# Autodesk Inventor assembly: Assembly_miniSPIM_v1
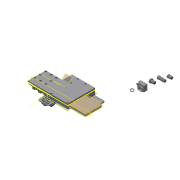
[picture p0: Inventor's stored thumbnail of the model, 180x180]
Saved by Autodesk Inventor 2019 (Build 230136000, 136)
## iProperties
Created: 2019-10-10
Part Number: Assembly_miniSPIM_v1
Document SubType Name: Assembly
Designer: diederichbenedict
Author: diederichbenedict
## Documents named in this file (19)
- C:\Users\diederichbenedict\Dropbox\Dokumente\Promotion\PROJECTS\miniSPIM\INVENTOR\Assembly_miniSPIM_v1.iam
- C:\Users\diederichbenedict\Dropbox\Dokumente\Promotion\PROJECTS\miniSPIM\INVENTOR\00_Huawei_P9.ipt
- C:\Users\diederichbenedict\Dropbox\Dokumente\Promotion\PROJECTS\miniSPIM\INVENTOR\00_Lens_f_25mm.ipt
- C:\Users\diederichbenedict\Dropbox\Dokumente\Promotion\PROJECTS\miniSPIM\INVENTOR\00_Sony_MDL_Projector.ipt
- C:\Users\diederichbenedict\Dropbox\Dokumente\Promotion\PROJECTS\miniSPIM\INVENTOR\00_XY_stage-CHUO_SEIKI_LD-647-R1.iam
- C:\Users\diederichbenedict\Dropbox\Dokumente\Promotion\PROJECTS\miniSPIM\INVENTOR\101_CCTV_Lens_Thread.ipt
- C:\Users\diederichbenedict\Dropbox\Dokumente\Promotion\PROJECTS\miniSPIM\INVENTOR\102_Z_Focus_CCTV_Camera.ipt
- C:\Users\diederichbenedict\Dropbox\Dokumente\Promotion\PROJECTS\miniSPIM\INVENTOR\103_CCTV_Lens_f2.8_f#1.ipt
- C:\Users\diederichbenedict\Dropbox\Dokumente\Promotion\PROJECTS\miniSPIM\INVENTOR\104_CCTV_Lens_f2.8_#1.ipt
- C:\Users\diederichbenedict\Dropbox\Dokumente\Promotion\PROJECTS\miniSPIM\INVENTOR\105_CCTV_Lens_f6_f#1.ipt
- C:\Users\diederichbenedict\Dropbox\Dokumente\Promotion\PROJECTS\miniSPIM\INVENTOR\00_Lightpath.ipt
- C:\Users\diederichbenedict\Dropbox\Dokumente\Promotion\PROJECTS\miniSPIM\INVENTOR\10_MiniSPIM_Base_v1.ipt
- C:\Users\diederichbenedict\Dropbox\Dokumente\Promotion\PROJECTS\miniSPIM\INVENTOR\00_Mirror_10mmDia.ipt
- C:\Users\diederichbenedict\Dropbox\Dokumente\Promotion\PROJECTS\miniSPIM\INVENTOR\10_MiniSPIM_Lid.ipt
- C:\Users\diederichbenedict\Dropbox\Dokumente\Promotion\PROJECTS\miniSPIM\INVENTOR\10_MiniSPIM_Smarthponebase.ipt
- C:\Users\diederichbenedict\Dropbox\Dokumente\Promotion\PROJECTS\miniSPIM\INVENTOR\10_MiniSPIM_Samplechamber.ipt
- C:\Users\diederichbenedict\Dropbox\Dokumente\Promotion\PROJECTS\miniSPIM\INVENTOR\10_MiniSPIM_Sampleholder.ipt
- C:\Users\diederichbenedict\Dropbox\Dokumente\Promotion\PROJECTS\miniSPIM\INVENTOR\00_XY-Tisch_Chinaware_Benedict-Diederich.ipt
- C:\Users\diederichbenedict\Dropbox\Dokumente\Promotion\PROJECTS\miniSPIM\INVENTOR\10_MiniSPIM_XY_Stageplate.ipt
## Components (19 placed, 18 different names)
1. 00_Huawei_P9:1 — Mate:1, Angle:1, Mate:2
2. 00_Lens_f_25mm:1 — Insert:1, Flush:4
3. 00_Sony_MDL_Projector:1 — Flush:1, Mate:1, Angle:1, Angle:2, Insert:1, Flush:3, Flush:5, Flush:6, Flush:9, Flush:10
4. 00_XY_stage-CHUO_SEIKI_LD-647-R1:1 [sub-assembly] — Flush:1, Angle:2, Flush:8, Flush:17, Flush:18, Mate:6, Mate:7, Flush:20, Flush:21
5. 101_CCTV_Lens_Thread:1
6. 102_Z_Focus_CCTV_Camera:1
7. 103_CCTV_Lens_f2.8_f#1:1
8. 104_CCTV_Lens_f2.8_#1:1
9. 105_CCTV_Lens_f6_f#1:1
10. 103_CCTV_Lens_f2.8_f#1:2 — Mate:3, Flush:7
11. 00_Lightpath:1 — Flush:3, Flush:4, Flush:5, Flush:6, Mate:2, Mate:3, Flush:7, Flush:8, Mate:4, Angle:3
12. 10_MiniSPIM_Base_v1:1 — Flush:9, Flush:10, Flush:11, Flush:12, Flush:15, Flush:16, Flush:19
13. 00_Mirror_10mmDia:1 — Mate:5
14. 10_MiniSPIM_Lid:1 — Flush:11, Flush:12, Flush:13, Flush:14
15. 10_MiniSPIM_Smarthponebase:1 — Flush:13, Flush:14
16. 10_MiniSPIM_Samplechamber:1 — Flush:15, Flush:16
17. 10_MiniSPIM_Sampleholder:1 — Flush:17, Flush:18
18. 00_XY-Tisch_Chinaware_Benedict-Diederich:1 — Mate:6, Flush:19, Mate:7
19. 10_MiniSPIM_XY_Stageplate:1 — Flush:20, Flush:21
## Relationships (31: Flush 20, Mate 7, Angle 3, Insert 1)
- Flush:1: 00_Sony_MDL_Projector:1 ↔ 00_XY_stage-CHUO_SEIKI_LD-647-R1:1
- Mate:1 (10 mm): 00_Huawei_P9:1 ↔ 00_Sony_MDL_Projector:1
- Angle:1 (0 deg): 00_Huawei_P9:1 ↔ 00_Sony_MDL_Projector:1
- Angle:2 (-90 deg): 00_Sony_MDL_Projector:1 ↔ 00_XY_stage-CHUO_SEIKI_LD-647-R1:1
- Insert:1 (-2 mm): 00_Lens_f_25mm:1 ↔ 00_Sony_MDL_Projector:1
- Flush:3: 00_Sony_MDL_Projector:1 ↔ 00_Lightpath:1
- Flush:4 (15 mm): 00_Lens_f_25mm:1 ↔ 00_Lightpath:1
- Flush:5: 00_Sony_MDL_Projector:1 ↔ 00_Lightpath:1
- Flush:6: 00_Sony_MDL_Projector:1 ↔ 00_Lightpath:1
- Mate:2: 00_Huawei_P9:1 ↔ 00_Lightpath:1
- Mate:3: 103_CCTV_Lens_f2.8_f#1:2 ↔ 00_Lightpath:1
- Flush:7 (6.7 mm): 103_CCTV_Lens_f2.8_f#1:2 ↔ 00_Lightpath:1
- Flush:8: 00_XY_stage-CHUO_SEIKI_LD-647-R1:1 ↔ 00_Lightpath:1
- Flush:9: 00_Sony_MDL_Projector:1 ↔ 10_MiniSPIM_Base_v1:1
- Flush:10 (3 mm): 00_Sony_MDL_Projector:1 ↔ 10_MiniSPIM_Base_v1:1
- Mate:4: 00_Lightpath:1
- Angle:3 (90 deg): 00_Lightpath:1
- Mate:5: 00_Mirror_10mmDia:1
- Flush:11: 10_MiniSPIM_Base_v1:1 ↔ 10_MiniSPIM_Lid:1
- Flush:12: 10_MiniSPIM_Base_v1:1 ↔ 10_MiniSPIM_Lid:1
- Flush:13: 10_MiniSPIM_Lid:1 ↔ 10_MiniSPIM_Smarthponebase:1
- Flush:14: 10_MiniSPIM_Lid:1 ↔ 10_MiniSPIM_Smarthponebase:1
- Flush:15: 10_MiniSPIM_Base_v1:1 ↔ 10_MiniSPIM_Samplechamber:1
- Flush:16: 10_MiniSPIM_Base_v1:1 ↔ 10_MiniSPIM_Samplechamber:1
- Flush:17: 00_XY_stage-CHUO_SEIKI_LD-647-R1:1 ↔ 10_MiniSPIM_Sampleholder:1
- Flush:18: 00_XY_stage-CHUO_SEIKI_LD-647-R1:1 ↔ 10_MiniSPIM_Sampleholder:1
- Mate:6 (5 mm): 00_XY_stage-CHUO_SEIKI_LD-647-R1:1 ↔ 00_XY-Tisch_Chinaware_Benedict-Diederich:1
- Flush:19: 10_MiniSPIM_Base_v1:1 ↔ 00_XY-Tisch_Chinaware_Benedict-Diederich:1
- Mate:7: 00_XY_stage-CHUO_SEIKI_LD-647-R1:1 ↔ 00_XY-Tisch_Chinaware_Benedict-Diederich:1
- Flush:20: 00_XY_stage-CHUO_SEIKI_LD-647-R1:1 ↔ 10_MiniSPIM_XY_Stageplate:1
- Flush:21: 00_XY_stage-CHUO_SEIKI_LD-647-R1:1 ↔ 10_MiniSPIM_XY_Stageplate:1
